# Autodesk Inventor assembly: Leg_joint_roll_pitch
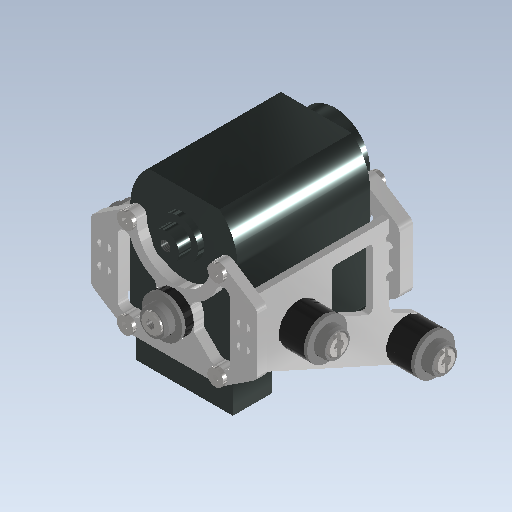
[picture p0: Inventor's stored thumbnail of the model, 512x512]
Saved by Autodesk Inventor 2020 (Build 240168000, 168)
## iProperties
Part Number: Leg_joint_roll_pitch
Document SubType Name: Assembly
Designer: Masato Kubotera
Mass: 155.537 g
Surface Area: 333.044 cm^2
Volume: 75.5065 cm^3
Density: 2.05992 g/cm^3
Author: Masato Kubotera
## Documents named in this file (17)
- C:\Users\Masato\Documents\Inventor\CIT Brains_Inventor\OpenPlatform_ver3_0\LowerBody\Leg_joit\Leg_joint_roll_pitch.iam
- C:\Users\Masato\Documents\Inventor\CIT Brains_Inventor\OpenPlatform_ver3_0\LowerBody\Leg_joit\Leg_joint_pitch_frame.ipt
- C:\Users\Masato\Documents\Inventor\CIT Brains_Inventor\OpenPlatform_ver3_0\LowerBody\Leg_joit\Leg_joint_roll_front_frame.ipt
- C:\Users\Masato\Documents\Inventor\CIT Brains_Inventor\OpenPlatform_ver3_0\Ready_Made\B3M11xx.ipt
- C:\Users\Masato\Documents\Inventor\CIT Brains_Inventor\OpenPlatform_ver3_0\Ready_Made\SLSBF6-39_5-M3-N3.ipt
- C:\Users\Masato\Documents\Inventor\CIT Brains_Inventor\OpenPlatform_ver3_0\Ready_Made\UUW-0312-10BH.ipt
- C:\Users\Masato\Documents\Inventor\CIT Brains_Inventor\OpenPlatform_ver3_0\Ready_Made\BRU-311S.ipt
- C:\Users\Masato\Documents\Inventor\CIT Brains_Inventor\OpenPlatform_ver3_0\Ready_Made\Screw\M2_6-20.ipt
- C:\Users\Masato\Documents\Inventor\CIT Brains_Inventor\OpenPlatform_ver3_0\Ready_Made\Screw\M2_6-15.ipt
- C:\Users\Masato\Documents\Inventor\CIT Brains_Inventor\OpenPlatform_ver3_0\Ready_Made\80F-0603.ipt
- C:\Users\Masato\Documents\Inventor\CIT Brains_Inventor\OpenPlatform_ver3_0\Ready_Made\CC-0612-15B.ipt
- C:\Users\Masato\Documents\Inventor\CIT Brains_Inventor\OpenPlatform_ver3_0\Ready_Made\CC-0612-50B.ipt
- C:\Users\Masato\Documents\Inventor\CIT Brains_Inventor\OpenPlatform_ver3_0\Ready_Made\SF319.ipt
- C:\Users\Masato\Documents\Inventor\CIT Brains_Inventor\OpenPlatform_ver3_0\Ready_Made\S3-07-3W.ipt
- C:\Users\Masato\Documents\Inventor\CIT Brains_Inventor\OpenPlatform_ver3_0\Ready_Made\ARU-306S.ipt
- C:\Users\Masato\Documents\Inventor\CIT Brains_Inventor\OpenPlatform_ver3_0\Ready_Made\BRU-307_5S.ipt
- C:\Users\Masato\Documents\Inventor\CIT Brains_Inventor\OpenPlatform_ver3_0\LowerBody\Leg_joit\Leg_joint_roll_back_frame.ipt
## Components (48 placed, 16 different names)
1. Leg_joint_pitch_frame:1 — フラッシュ:1, 挿入:11, 挿入:27, 挿入:28, 挿入:133
2. Leg_joint_pitch_frame:2 — 挿入:12, 挿入:25, 挿入:26, フラッシュ:1, 挿入:132, メイト:11, メイト:12, フラッシュ:7
3. B3M11xx:1 — フラッシュ:6, メイト:8, メイト:10, 挿入:152, 挿入:153, 挿入:154, 挿入:155, 挿入:180, 挿入:181, 挿入:182, 挿入:183
4. SLSBF6-39_5-M3-N3:1 — 挿入:11, 挿入:12
5. UUW-0312-10BH:1 — 挿入:27, 挿入:100, 挿入:124
6. UUW-0312-10BH:2 — 挿入:28, 挿入:101, 挿入:125
7. UUW-0312-10BH:3 — 挿入:25, 挿入:99, 挿入:126
8. UUW-0312-10BH:4 — 挿入:26, 挿入:98, 挿入:127
9. UUW-0312-10BH:5 — 挿入:175, 挿入:188
10. UUW-0312-10BH:6 — 挿入:120, 挿入:156, 挿入:171
11. BRU-311S:1 — 挿入:99
12. BRU-311S:2 — 挿入:98
13. BRU-311S:3 — 挿入:101
14. BRU-311S:4 — 挿入:100
15. M2_6-20:1 — 挿入:157
16. M2_6-20:2 — 挿入:159
17. M2_6-20:3 — 挿入:158
18. M2_6-20:4 — 挿入:160
19. M2_6-15:1 — 挿入:184
20. M2_6-15:2 — 挿入:185
21. M2_6-15:3 — 挿入:186
22. M2_6-15:4 — 挿入:187
23. 80F-0603:1 — 挿入:134
24. 80F-0603:3 — 挿入:130
25. 80F-0603:4 — 挿入:131
26. 80F-0603:5 — 挿入:129
27. 80F-0603:6 — 挿入:128
28. CC-0612-15B:1 — 挿入:114, 挿入:124
29. CC-0612-15B:2 — 挿入:115, 挿入:125
30. CC-0612-15B:3 — 挿入:116, 挿入:127
31. CC-0612-15B:4 — 挿入:117, 挿入:126
32. CC-0612-15B:5 — 挿入:120, 挿入:134
33. CC-0612-50B:1 — 挿入:114, 挿入:130
34. CC-0612-50B:2 — 挿入:115, 挿入:131
35. CC-0612-50B:3 — 挿入:116, 挿入:128
36. CC-0612-50B:4 — 挿入:117, 挿入:129
37. SF319:1 — 挿入:132
38. SF319:2 — 挿入:133
39. S3-07-3W:1 — 角度:1, 挿入:151
40. Leg_joint_roll_front_frame:1 — 角度:1, 挿入:151, 挿入:152, 挿入:153, 挿入:154, 挿入:155, 挿入:156, 挿入:157, 挿入:158, 挿入:159, 挿入:160, メイト:11, メイト:12, フラッシュ:7
41. ARU-306S:1 — 挿入:171
42. 80F-0603:7 — 挿入:179
43. BRU-307_5S:1 — 挿入:189
44. Leg_joint_roll_back_frame:1 — 角度:2, 挿入:174, 挿入:175, 挿入:180, 挿入:181, 挿入:182, 挿入:183, 挿入:184, 挿入:185, 挿入:186, 挿入:187
45. S3-07-3W:2 — 角度:2, 挿入:174
46. CC-0612-15B:6 — 挿入:178, 挿入:190
47. CC-0612-15B:7 — 挿入:178, 挿入:179
48. UUW-0312-10BH:7 — 挿入:188, 挿入:189, 挿入:190
## Relationships (61: Insert 52, Mate 4, Flush 3, Angle 2)
- フラッシュ:1 [Flush]: Leg_joint_pitch_frame:1 ↔ Leg_joint_pitch_frame:2
- 挿入:11 [Insert]: Leg_joint_pitch_frame:1 ↔ SLSBF6-39_5-M3-N3:1
- 挿入:12 [Insert]: Leg_joint_pitch_frame:2 ↔ SLSBF6-39_5-M3-N3:1
- 挿入:25 [Insert]: Leg_joint_pitch_frame:2 ↔ UUW-0312-10BH:3
- 挿入:26 [Insert]: Leg_joint_pitch_frame:2 ↔ UUW-0312-10BH:4
- 挿入:27 [Insert]: Leg_joint_pitch_frame:1 ↔ UUW-0312-10BH:1
- 挿入:28 [Insert]: Leg_joint_pitch_frame:1 ↔ UUW-0312-10BH:2
- フラッシュ:6 [Flush]: B3M11xx:1
- メイト:8 [Mate]: B3M11xx:1
- メイト:10 [Mate]: B3M11xx:1
- 挿入:98 [Insert]: UUW-0312-10BH:4 ↔ BRU-311S:2
- 挿入:99 [Insert]: UUW-0312-10BH:3 ↔ BRU-311S:1
- 挿入:100 [Insert]: UUW-0312-10BH:1 ↔ BRU-311S:4
- 挿入:101 [Insert]: UUW-0312-10BH:2 ↔ BRU-311S:3
- 挿入:114 [Insert]: CC-0612-15B:1 ↔ CC-0612-50B:1
- 挿入:115 [Insert]: CC-0612-15B:2 ↔ CC-0612-50B:2
- 挿入:116 [Insert]: CC-0612-15B:3 ↔ CC-0612-50B:3
- 挿入:117 [Insert]: CC-0612-15B:4 ↔ CC-0612-50B:4
- 挿入:120 [Insert]: UUW-0312-10BH:6 ↔ CC-0612-15B:5
- 挿入:124 [Insert]: UUW-0312-10BH:1 ↔ CC-0612-15B:1
- 挿入:125 [Insert]: UUW-0312-10BH:2 ↔ CC-0612-15B:2
- 挿入:126 [Insert]: UUW-0312-10BH:3 ↔ CC-0612-15B:4
- 挿入:127 [Insert]: UUW-0312-10BH:4 ↔ CC-0612-15B:3
- 挿入:128 [Insert]: 80F-0603:6 ↔ CC-0612-50B:3
- 挿入:129 [Insert]: 80F-0603:5 ↔ CC-0612-50B:4
- 挿入:130 [Insert]: 80F-0603:3 ↔ CC-0612-50B:1
- 挿入:131 [Insert]: 80F-0603:4 ↔ CC-0612-50B:2
- 挿入:132 [Insert]: Leg_joint_pitch_frame:2 ↔ SF319:1
- 挿入:133 [Insert]: Leg_joint_pitch_frame:1 ↔ SF319:2
- 挿入:134 [Insert]: 80F-0603:1 ↔ CC-0612-15B:5
- 角度:1 [Angle] (0 deg): S3-07-3W:1 ↔ Leg_joint_roll_front_frame:1
- 挿入:151 [Insert]: S3-07-3W:1 ↔ Leg_joint_roll_front_frame:1
- 挿入:152 [Insert]: B3M11xx:1 ↔ Leg_joint_roll_front_frame:1
- 挿入:153 [Insert]: B3M11xx:1 ↔ Leg_joint_roll_front_frame:1
- 挿入:154 [Insert]: B3M11xx:1 ↔ Leg_joint_roll_front_frame:1
- 挿入:155 [Insert]: B3M11xx:1 ↔ Leg_joint_roll_front_frame:1
- 挿入:156 [Insert]: UUW-0312-10BH:6 ↔ Leg_joint_roll_front_frame:1
- 挿入:157 [Insert]: M2_6-20:1 ↔ Leg_joint_roll_front_frame:1
- 挿入:158 [Insert]: M2_6-20:3 ↔ Leg_joint_roll_front_frame:1
- 挿入:159 [Insert]: M2_6-20:2 ↔ Leg_joint_roll_front_frame:1
- 挿入:160 [Insert]: M2_6-20:4 ↔ Leg_joint_roll_front_frame:1
- メイト:11 [Mate] (0.01 mm): Leg_joint_pitch_frame:2 ↔ Leg_joint_roll_front_frame:1
- メイト:12 [Mate] (0.01 mm): Leg_joint_pitch_frame:2 ↔ Leg_joint_roll_front_frame:1
- フラッシュ:7 [Flush]: Leg_joint_pitch_frame:2 ↔ Leg_joint_roll_front_frame:1
- 挿入:171 [Insert]: UUW-0312-10BH:6 ↔ ARU-306S:1
- 角度:2 [Angle] (0 deg): Leg_joint_roll_back_frame:1 ↔ S3-07-3W:2
- 挿入:174 [Insert]: Leg_joint_roll_back_frame:1 ↔ S3-07-3W:2
- 挿入:175 [Insert]: UUW-0312-10BH:5 ↔ Leg_joint_roll_back_frame:1
- 挿入:178 [Insert]: CC-0612-15B:6 ↔ CC-0612-15B:7
- 挿入:179 [Insert]: 80F-0603:7 ↔ CC-0612-15B:7
- 挿入:180 [Insert]: B3M11xx:1 ↔ Leg_joint_roll_back_frame:1
- 挿入:181 [Insert]: B3M11xx:1 ↔ Leg_joint_roll_back_frame:1
- 挿入:182 [Insert]: B3M11xx:1 ↔ Leg_joint_roll_back_frame:1
- 挿入:183 [Insert]: B3M11xx:1 ↔ Leg_joint_roll_back_frame:1
- 挿入:184 [Insert]: M2_6-15:1 ↔ Leg_joint_roll_back_frame:1
- 挿入:185 [Insert]: M2_6-15:2 ↔ Leg_joint_roll_back_frame:1
- 挿入:186 [Insert]: M2_6-15:3 ↔ Leg_joint_roll_back_frame:1
- 挿入:187 [Insert]: M2_6-15:4 ↔ Leg_joint_roll_back_frame:1
- 挿入:188 [Insert]: UUW-0312-10BH:5 ↔ UUW-0312-10BH:7
- 挿入:189 [Insert]: BRU-307_5S:1 ↔ UUW-0312-10BH:7
- 挿入:190 [Insert]: CC-0612-15B:6 ↔ UUW-0312-10BH:7
